# Autodesk Inventor assembly: Inner Bracket
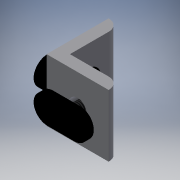
[picture p0: Inventor's stored thumbnail of the model, 180x180]
Saved by Autodesk Inventor 2019 (Build 230136000, 136)
## iProperties
Created: 2018-10-13
Part Number: Inner Bracket
Document SubType Name: Assembly
Designer: nomol
Author: nomol
## Documents named in this file (4)
- C:\Users\nomol\Downloads\Inventor\Helmholtz Cage\Inner Bracket.iam
- C:\Users\nomol\Downloads\Inventor\Helmholtz Cage\8020_CornerBracket.ipt
- C:\Users\nomol\Downloads\Inventor\Helmholtz Cage\8020_SlideInTNut.ipt
- C:\Users\nomol\Downloads\Inventor\Helmholtz Cage\8020_ButtonScrewMedium.ipt
## Components (5 placed, 3 different names)
1. 8020_CornerBracket:1 — Insert:1, Insert:3
2. 8020_SlideInTNut:1 — Insert:1, Insert:2
3. 8020_SlideInTNut:2 — Insert:3, Insert:4
4. 8020_ButtonScrewMedium:1 — Insert:4
5. 8020_ButtonScrewMedium:2 — Insert:2
## Relationships (4: Insert 4)
- Insert:1 (4.5 mm): 8020_CornerBracket:1 ↔ 8020_SlideInTNut:1
- Insert:2: 8020_SlideInTNut:1 ↔ 8020_ButtonScrewMedium:2
- Insert:3 (4.5 mm): 8020_CornerBracket:1 ↔ 8020_SlideInTNut:2
- Insert:4: 8020_SlideInTNut:2 ↔ 8020_ButtonScrewMedium:1
